# Autodesk Inventor assembly: A2017_T2_02
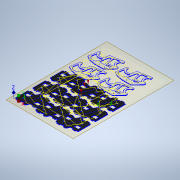
[picture p0: Inventor's stored thumbnail of the model, 180x180]
Saved by Autodesk Inventor 2022 (Build 260153000, 153)
## iProperties
Created: 2022-09-28
Part Number: A2017_T2_02
Document SubType Name: Assembly
Designer: Masato
Author: Masato
## Documents named in this file (4)
- C:\Users\6343y\ドキュメント\Inventor\SUSTAINA-OP\Cam\A2017_T2\A2017_T2_03.iam
- C:\Users\6343y\ドキュメント\Inventor\SUSTAINA-OP\Cam\DisposableBoard.ipt
- C:\Users\6343y\ドキュメント\Inventor\SUSTAINA-OP\LowerBody\Leg_joint\Leg_joint_pitch_frame.ipt
- C:\Users\6343y\ドキュメント\Inventor\SUSTAINA-OP\LowerBody\Knee\Knee_side_frame.ipt
## Components (23 placed, 3 different names)
1. DisposableBoard:1 — フラッシュ:1, フラッシュ:2, フラッシュ:3, フラッシュ:4, フラッシュ:5, 正接:1, フラッシュ:6, 正接:2
2. Leg_joint_pitch_frame:1 — メイト:1, メイト:3, 正接:1
3. Leg_joint_pitch_frame:2 — メイト:2, メイト:3, フラッシュ:5, フラッシュ:6
4. Leg_joint_pitch_frame:3
5. Leg_joint_pitch_frame:4
6. Leg_joint_pitch_frame:5
7. Leg_joint_pitch_frame:6
8. Leg_joint_pitch_frame:7
9. Leg_joint_pitch_frame:8
10. Leg_joint_pitch_frame:9
11. Leg_joint_pitch_frame:10
12. Leg_joint_pitch_frame:11
13. Leg_joint_pitch_frame:12
14. Leg_joint_pitch_frame:13 — メイト:5
15. Leg_joint_pitch_frame:14
16. Leg_joint_pitch_frame:15
17. Leg_joint_pitch_frame:16
18. Leg_joint_pitch_frame:17
19. Leg_joint_pitch_frame:18
20. Knee_side_frame:1 — メイト:4, メイト:5, 正接:2
21. Knee_side_frame:2
22. Knee_side_frame:3
23. Knee_side_frame:4
## Component patterns: (9 elements, first: Leg_joint_pitch_frame:1 + Leg_joint_pitch_frame:2), (4 elements, first: Knee_side_frame:1)
## Relationships (13: Flush 6, Mate 5, Tangent 2)
- フラッシュ:1 [Flush]: DisposableBoard:1
- フラッシュ:2 [Flush]: DisposableBoard:1
- フラッシュ:3 [Flush]: DisposableBoard:1
- フラッシュ:4 [Flush]: DisposableBoard:1
- メイト:1 [Mate]: Leg_joint_pitch_frame:1
- メイト:2 [Mate]: Leg_joint_pitch_frame:2
- メイト:3 [Mate] (2.1 mm): Leg_joint_pitch_frame:1 ↔ Leg_joint_pitch_frame:2
- フラッシュ:5 [Flush] (2.1 mm): DisposableBoard:1 ↔ Leg_joint_pitch_frame:2
- 正接:1 [Tangent] (2.1 mm): DisposableBoard:1 ↔ Leg_joint_pitch_frame:1
- フラッシュ:6 [Flush] (2.1 mm): DisposableBoard:1 ↔ Leg_joint_pitch_frame:2
- メイト:4 [Mate]: Knee_side_frame:1
- メイト:5 [Mate] (2.1 mm): Leg_joint_pitch_frame:13 ↔ Knee_side_frame:1
- 正接:2 [Tangent] (2.1 mm): DisposableBoard:1 ↔ Knee_side_frame:1
